# Autodesk Inventor assembly: frameortho
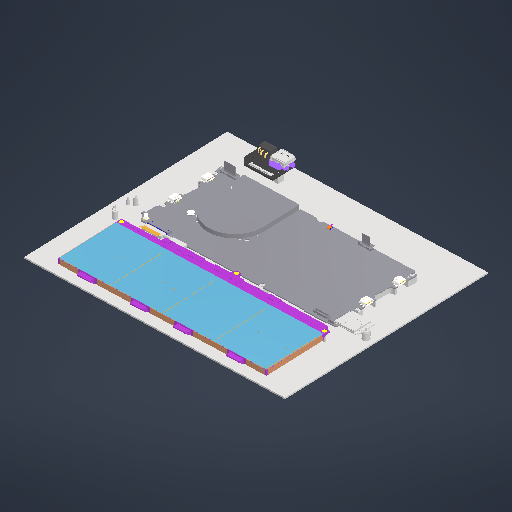
[picture p0: Inventor's stored thumbnail of the model, 512x512]
Saved by Autodesk Inventor 2026.2 (Build 302298000, 298)
## iProperties
Created: 2026-01-15
Part Number: frameortho
Document SubType Name: Assembly
Designer: 200481997
Author: 200481997
## Documents named in this file (6)
- C:\Users\chinh\Documents\frameergo\CAD\frameergo.iam
- C:\Users\chinh\Documents\frameergo\CAD\Imports\Battery\FWKNAQ9_G01_20210911\Framework BatteryFWKNAQ9_G01_20210911.ipt
- C:\Users\chinh\Documents\frameergo\CAD\chassis.ipt
- C:\Users\chinh\Documents\frameergo\CAD\Imports\Motherboard\Framework Mobo\Framework Mobo.ipt
- C:\Users\chinh\Documents\frameergo\CAD\Imports\DisplayPort Adapter\source\source.ipt
- C:\Users\chinh\Documents\frameergo\CAD\Imports\Wifi Card\3D Model - MT320, M.2 2230, Key E, SDIO (453-00178)\3D Model - MT320, M.2 2230, Key E, SDIO (453-00178).ipt
## Components (5 placed, 5 different names)
1. Framework Battery — Mate:5
2. Frameergo Chassis — Mate:1, Mate:2, Mate:3, Mate:4, Mate:5, Rotational:1
3. Framework Mobo — Mate:1, Mate:2, Angle:1
4. DisplayPort Source Adapter — Mate:3, Mate:4
5. 3D Model - MT320, M.2 2230, Key E, SDIO (453-00178):1 — Rotational:1, Angle:1
## Relationships (7: Mate 5, RevoluteJoint 1, Angle 1)
- Mate:1: Frameergo Chassis ↔ Framework Mobo
- Mate:2: Frameergo Chassis ↔ Framework Mobo
- Mate:3: Frameergo Chassis ↔ DisplayPort Source Adapter
- Mate:4: Frameergo Chassis ↔ DisplayPort Source Adapter
- Mate:5: Framework Battery ↔ Frameergo Chassis
- Rotational:1 [RevoluteJoint]: Frameergo Chassis ↔ 3D Model - MT320, M.2 2230, Key E, SDIO (453-00178):1
- Angle:1 (180 deg): Framework Mobo ↔ 3D Model - MT320, M.2 2230, Key E, SDIO (453-00178):1
